# Autodesk Inventor assembly: Case
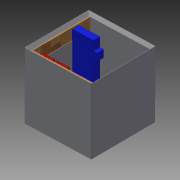
[picture p0: Inventor's stored thumbnail of the model, 180x180]
Saved by Autodesk Inventor 2015 (Build 190159000, 159)
## iProperties
Created: 2016-03-23
Part Number: Case
Document SubType Name: Assembly
Designer: Noah
Author: Noah
## Documents named in this file (17)
- C:\Users\Noah\Projects\PC_Cube\Case.iam
- C:\Users\Noah\Projects\PC_Cube\Bot.ipt
- C:\Users\Noah\Projects\PC_Cube\Top.ipt
- C:\Users\Noah\Projects\PC_Cube\Back.ipt
- C:\Users\Noah\Projects\PC_Cube\Front.ipt
- C:\Users\Noah\Projects\PC_Cube\Left.ipt
- C:\Users\Noah\Projects\PC_Cube\Right.ipt
- C:\Users\Noah\Projects\PC_Cube\Parameters.ipt
- C:\Users\Noah\Projects\PC_Cube\PSU.ipt
- C:\Users\Noah\Projects\PC_Cube\SSD2.5.ipt
- C:\Users\Noah\Projects\PC_Cube\HDD3.5.ipt
- C:\Users\Noah\Projects\PC_Cube\Side_left.ipt
- C:\Users\Noah\Projects\PC_Cube\Mobo.ipt
- C:\Users\Noah\Projects\PC_Cube\Side_back.ipt
- C:\Users\Noah\Projects\PC_Cube\Fan120mm.ipt
- C:\Users\Noah\Projects\PC_Cube\Arrow.ipt
- C:\Users\Noah\Projects\PC_Cube\Foot.ipt
## Components (22 placed, 16 different names)
1. Top:1 — Mate:45, Mate:46, Mate:47, Mate:48
2. Back:1 — Angle:1, Mate:41, Mate:42, Mate:46, Mate:54
3. Front:1 — Mate:37, Mate:40, Mate:43, Mate:44, Mate:45, Mate:55, Mate:56
4. Left:1 — Mate:16, Mate:36, Mate:42, Mate:43, Mate:48, Mate:58
5. Right:1 — Angle:1, Mate:41, Mate:44, Mate:47, Mate:53, Mate:57
6. Parameters:1
7. PSU:1 — Mate:26, Mate:27, Flush:21, Mate:34
8. SSD2.5:1 — Flush:15, Flush:16, Mate:21, Flush:19
9. SSD2.5:2 — Flush:15, Flush:16, Mate:21, Mate:24, Flush:20
10. HDD3.5:1 — Flush:17, Flush:18, Mate:22, Mate:23, Mate:25, Flush:20
11. HDD3.5:2 — Flush:17, Flush:18, Mate:22, Mate:34
12. Side_left:1 — Mate:16, Mate:17, Flush:10, Mate:18, Flush:11, Flush:13, Mate:20, Flush:28, Mate:36
13. Mobo:1 — Mate:17, Mate:20, Flush:14, Mate:29, Flush:28
14. Side_back:1 — Flush:10, Mate:18, Flush:11, Mate:19, Flush:12, Mate:23, Mate:24, Flush:19, Mate:27, Flush:21, Mate:37, Mate:40
15. Bot:2 — Mate:19, Flush:12, Flush:13, Flush:14, Mate:25, Mate:26, Flush:22, Mate:28, Flush:26, Flush:27, Flush:30, Mate:50, Mate:51, Mate:52
16. Fan120mm:1 — Flush:22, Flush:26, Flush:27, Mate:35, Flush:29, Mate:39
17. Fan120mm:2 — Mate:28, Mate:29, Mate:35, Mate:38, Mate:49
18. Arrow:3 — Flush:29, Mate:39
19. Arrow:4 — Mate:38, Mate:49
20. Foot:1 — Flush:30, Mate:50, Mate:53, Mate:54
21. Foot:2 — Mate:51, Mate:55, Mate:57
22. Foot:3 — Mate:52, Mate:56, Mate:58
## Relationships (58: Mate 39, Flush 18, Angle 1)
- Mate:16: Left:1 ↔ Side_left:1
- Mate:17: Side_left:1 ↔ Mobo:1
- Flush:10: Side_left:1 ↔ Side_back:1
- Mate:18: Side_left:1 ↔ Side_back:1
- Flush:11: Side_left:1 ↔ Side_back:1
- Mate:19: Side_back:1 ↔ Bot:2
- Flush:12: Side_back:1 ↔ Bot:2
- Flush:13: Side_left:1 ↔ Bot:2
- Mate:20: Side_left:1 ↔ Mobo:1
- Flush:14: Mobo:1 ↔ Bot:2
- Flush:15: SSD2.5:1 ↔ SSD2.5:2
- Flush:16: SSD2.5:1 ↔ SSD2.5:2
- Mate:21 (10 mm): SSD2.5:1 ↔ SSD2.5:2
- Flush:17: HDD3.5:1 ↔ HDD3.5:2
- Flush:18: HDD3.5:1 ↔ HDD3.5:2
- Mate:22 (10 mm): HDD3.5:1 ↔ HDD3.5:2
- Mate:23: HDD3.5:1 ↔ Side_back:1
- Mate:24: SSD2.5:2 ↔ Side_back:1
- Mate:25: HDD3.5:1 ↔ Bot:2
- Flush:19: SSD2.5:1 ↔ Side_back:1
- Flush:20: SSD2.5:2 ↔ HDD3.5:1
- Mate:26: PSU:1 ↔ Bot:2
- Mate:27: PSU:1 ↔ Side_back:1
- Flush:21: PSU:1 ↔ Side_back:1
- Flush:22: Bot:2 ↔ Fan120mm:1
- Mate:28: Bot:2 ↔ Fan120mm:2
- Mate:29 (50 mm): Mobo:1 ↔ Fan120mm:2
- Mate:34 (20 mm): PSU:1 ↔ HDD3.5:2
- Flush:26 (10 mm): Bot:2 ↔ Fan120mm:1
- Flush:27 (10 mm): Bot:2 ↔ Fan120mm:1
- Mate:35 (10 mm): Fan120mm:1 ↔ Fan120mm:2
- Flush:28 (20 mm): Side_left:1 ↔ Mobo:1
- Mate:36: Left:1 ↔ Side_left:1
- Mate:37: Front:1 ↔ Side_back:1
- Flush:29 (-90 mm): Fan120mm:1 ↔ Arrow:3
- Mate:38: Fan120mm:2 ↔ Arrow:4
- Mate:39: Fan120mm:1 ↔ Arrow:3
- Mate:40: Front:1 ↔ Side_back:1
- Angle:1 (270 deg): Back:1 ↔ Right:1
- Mate:41: Back:1 ↔ Right:1
- Mate:42: Back:1 ↔ Left:1
- Mate:43: Front:1 ↔ Left:1
- Mate:44: Front:1 ↔ Right:1
- Mate:45: Top:1 ↔ Front:1
- Mate:46: Top:1 ↔ Back:1
- Mate:47: Top:1 ↔ Right:1
- Mate:48: Top:1 ↔ Left:1
- Mate:49: Fan120mm:2 ↔ Arrow:4
- Flush:30: Bot:2 ↔ Foot:1
- Mate:50: Bot:2 ↔ Foot:1
- Mate:51: Bot:2 ↔ Foot:2
- Mate:52: Bot:2 ↔ Foot:3
- Mate:53 (144 mm): Right:1 ↔ Foot:1
- Mate:54 (50 mm): Back:1 ↔ Foot:1
- Mate:55 (50 mm): Front:1 ↔ Foot:2
- Mate:56 (50 mm): Front:1 ↔ Foot:3
- Mate:57 (80 mm): Right:1 ↔ Foot:2
- Mate:58 (80 mm): Left:1 ↔ Foot:3
## Named parameters: edge_length = 360 mm, wall_width = 16 mm, chamfer_outer = 2 mm
